# Autodesk Inventor assembly: White Knight
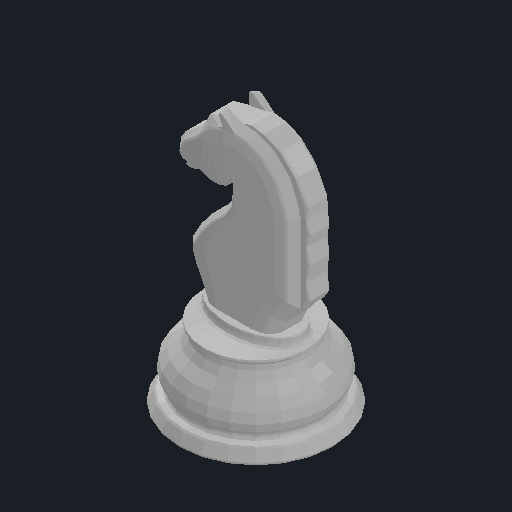
[picture p0: Inventor's stored thumbnail of the model, 512x512]
Saved by Autodesk Inventor 2026 (Build 300175000, 175)
## iProperties
Created: 2025-04-16
Part Number: White Knight
Document SubType Name: Assembly
Designer: ckyiu
Author: ckyiu
## Documents named in this file (3)
- C:\Users\ckyiu\Documents\Projects\Chessboard-Design\Assemblies\Chess Pieces\Black Knight.iam
- C:\Users\ckyiu\Documents\Projects\Chessboard-Design\Parts\Chess Pieces\White Knight.ipt
- C:\Users\ckyiu\Documents\Projects\Chessboard-Design\Parts\Generic Neodynium Magnet 10mm diameter 2mm height.ipt
## Components (2 placed, 2 different names)
1. White Knight:1 — Insert:1
2. Generic Neodynium Magnet 10mm diameter 2mm height:1 — Insert:1
## Relationships (1: Insert 1)
- Insert:1: White Knight:1 ↔ Generic Neodynium Magnet 10mm diameter 2mm height:1
